# Autodesk Inventor assembly: Assembly3
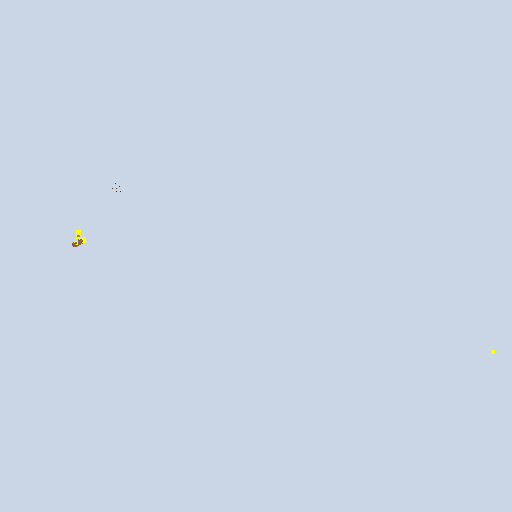
[picture p0: Inventor's stored thumbnail of the model, 512x512]
Saved by Autodesk Inventor 2024.1 (Build 281209000, 209)
## iProperties
Created: 2023-11-10
Part Number: Assembly3
Document SubType Name: Assembly
Designer: luvag
Author: luvag
## Documents named in this file (3)
- C:\Users\luvag\Desktop\Assembly3.iam
- C:\Users\luvag\Desktop\Assembly op.iam
- C:\Users\luvag\Desktop\Cannon.ipt
## Components (2 placed, 2 different names)
1. Assembly op:1 [sub-assembly]
2. Cannon:1
## Relationships (2: Mate 2)
- [Mate]: Assembly op:1 ↔ Cannon:1
- [Mate]: Assembly op:1 ↔ Cannon:1
